# Autodesk Inventor assembly: Assembly1
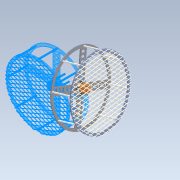
[picture p0: Inventor's stored thumbnail of the model, 180x180]
Saved by Autodesk Inventor 2021.1 (Build 251245010, 245A)
## iProperties
Created: 2023-10-20
Part Number: Assembly1
Document SubType Name: Assembly
Designer: Lenovo
Mass: 190.311 g
Surface Area: 1332.05 cm^2
Volume: 100.405 cm^3
Density: 1.89544 g/cm^3
Author: Lenovo
## Documents named in this file (4)
- F:\College\Semester_10\GP2\2DOF\2DOF_Hover\CAD\Workspaces\Workspace\Assembly1.iam
- F:\College\Semester_10\GP2\2DOF\2DOF_Hover\CAD\Workspaces\Workspace\Standoff M3 M-M H 45mm.ipt
- F:\College\Semester_10\GP2\2DOF\2DOF_Hover\CAD\Workspaces\Workspace\guard.ipt
- F:\College\Semester_10\GP2\2DOF\2DOF_Hover\CAD\Workspaces\Workspace\MotorWithPropeller.iam
## Components (6 placed, 3 different names)
1. Standoff M3 M-M H 45mm:1 — Mate:33, Mate:34
2. Standoff M3 M-M H 45mm:2 — Mate:31, Mate:32
3. Standoff M3 M-M H 45mm:3 — Mate:35, Mate:36
4. Standoff M3 M-M H 45mm:4 — Mate:37, Mate:38
5. guard:1 — Mate:31, Mate:32, Mate:33, Mate:34, Mate:35, Mate:36, Mate:37, Mate:38
6. MotorWithPropeller:1 [sub-assembly]
## Relationships (11: Mate 11)
- [Mate]: guard:1 ↔ MotorWithPropeller:1
- [Mate]: guard:1 ↔ MotorWithPropeller:1
- [Mate]: guard:1 ↔ MotorWithPropeller:1
- Mate:31: Standoff M3 M-M H 45mm:2 ↔ guard:1
- Mate:32: Standoff M3 M-M H 45mm:2 ↔ guard:1
- Mate:33: Standoff M3 M-M H 45mm:1 ↔ guard:1
- Mate:34: Standoff M3 M-M H 45mm:1 ↔ guard:1
- Mate:35: Standoff M3 M-M H 45mm:3 ↔ guard:1
- Mate:36: Standoff M3 M-M H 45mm:3 ↔ guard:1
- Mate:37: Standoff M3 M-M H 45mm:4 ↔ guard:1
- Mate:38: Standoff M3 M-M H 45mm:4 ↔ guard:1
